# Autodesk Inventor assembly: shin_bracket_assem
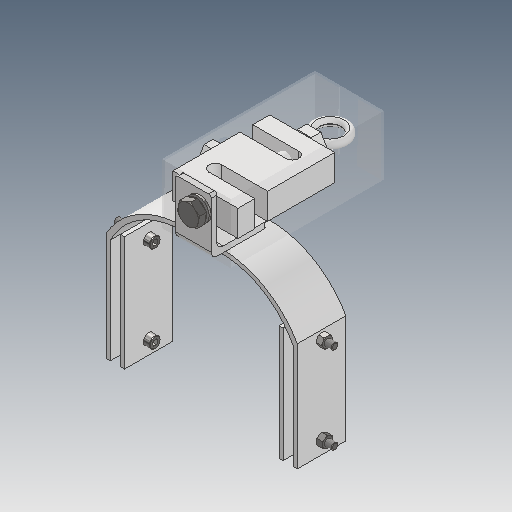
[picture p0: Inventor's stored thumbnail of the model, 512x512]
Saved by Autodesk Inventor 2025.2 (Build 292293000, 293)
## iProperties
Created: 2025-02-16
Part Number: shin_bracket_assem
Document SubType Name: Assembly
Designer: email
Author: email
## Documents named in this file (12)
- C:\Users\email\Desktop\Projects\Capstone\4TB6\CAD_Model\thigh_mount_2\shin_bracket_assem.iam
- C:\Users\email\Desktop\Projects\Capstone\4TB6\CAD_Model\thigh_mount_2\shin_bracket.ipt
- C:\Users\email\Desktop\Projects\Capstone\4TB6\CAD_Model\thigh_mount_2\shin_tab.ipt
- C:\Users\email\Documents\Inventor\Content Center Files\R2025\en-US\CSN 02 1143  A\CSN 02 1143 - M5 x 0.8 x 25(1).ipt
- C:\Users\email\Documents\Inventor\Content Center Files\R2025\en-US\AS 1112 (2)\AS 1112 - M5  Type 5.ipt
- C:\Users\email\Desktop\Projects\Capstone\4TB6\CAD_Model\thigh_mount_2\shin_L_bracket.ipt
- C:\Users\email\Documents\Inventor\Content Center Files\R2025\en-US\AS 1237 (2.1)\AS 1237 - 10.ipt
- C:\Users\email\Documents\Inventor\Content Center Files\R2025\en-US\AS 1110\AS 1110 - M10 x 16.ipt
- C:\Users\email\Documents\Inventor\Content Center Files\R2025\en-US\AS 1112 (2)\AS 1112 - M10  Type 5.ipt
- C:\Users\email\Desktop\Projects\Capstone\4TB6\CAD_Model\thigh_mount_2\tension_sensor_bolty.ipt
- C:\Users\email\Desktop\Projects\Capstone\4TB6\CAD_Model\thigh_mount_2\tension_sensor.ipt
- C:\Users\email\Desktop\Projects\Capstone\4TB6\CAD_Model\thigh_mount_2\tension_sensor_cover.ipt
## Components (21 placed, 11 different names)
1. shin_bracket:1 — Mate:2, Mate:3, Mate:11, Mate:12, Mate:13, Mate:14, Mate:19, Mate:20, Mate:21, Mate:22, Mate:23, Mate:24, Mate:26, Mate:28, Angle:1
2. shin_tab:1 — Mate:1, Mate:4, Mate:5, Mate:6, Mate:14
3. shin_tab:2 — Mate:7, Mate:8, Mate:9, Mate:10, Mate:13
4. CSN 02 1143 A M5 x 25:1 — Mate:1, Mate:2, Mate:5, Mate:17
5. CSN 02 1143 A M5 x 25:2 — Mate:3, Mate:4, Mate:6, Mate:18
6. CSN 02 1143 A M5 x 25:3 — Mate:7, Mate:9, Mate:11, Mate:15
7. CSN 02 1143 A M5 x 25:4 — Mate:8, Mate:10, Mate:12, Mate:16
8. AS 1112 (2) - Metric M5  Type 5:1 — Mate:16, Mate:20
9. AS 1112 (2) - Metric M5  Type 5:2 — Mate:15, Mate:19
10. AS 1112 (2) - Metric M5  Type 5:3 — Mate:17, Mate:21
11. AS 1112 (2) - Metric M5  Type 5:4 — Mate:18, Mate:22
12. shin_L_bracket:1 — Mate:23, Mate:24, Mate:30, Mate:31, Mate:32, Mate:33, Mate:36, Angle:1, Angle:2
13. AS 1237 (2.1) 10:1 — Mate:25, Mate:27, Mate:28
14. AS 1110 - Metric M10 x 16:1 — Mate:25, Mate:26, Mate:27, Mate:29
15. AS 1112 (2) - Metric M10  Type 5:1 — Mate:29, Mate:30
16. tension_sensor_bolty:1 — Mate:37, Mate:38, Mate:39
17. tension_sensor:1 — Mate:31, Mate:32, Mate:37, Mate:40, Angle:2
18. AS 1110 - Metric M10 x 16:2 — Mate:33, Mate:35, Mate:41, Mate:42
19. AS 1237 (2.1) 10:2 — Mate:35, Mate:36, Mate:43
20. AS 1237 (2.1) 10:3 — Mate:38, Mate:39, Mate:40
21. tension_sensor_cover:1 — Mate:41, Mate:42, Mate:43
## Relationships (44: Mate 42, Angle 2)
- Mate:1: shin_tab:1 ↔ CSN 02 1143 A M5 x 25:1
- Mate:2: shin_bracket:1 ↔ CSN 02 1143 A M5 x 25:1
- Mate:3: shin_bracket:1 ↔ CSN 02 1143 A M5 x 25:2
- Mate:4: shin_tab:1 ↔ CSN 02 1143 A M5 x 25:2
- Mate:5: shin_tab:1 ↔ CSN 02 1143 A M5 x 25:1
- Mate:6: shin_tab:1 ↔ CSN 02 1143 A M5 x 25:2
- Mate:7: shin_tab:2 ↔ CSN 02 1143 A M5 x 25:3
- Mate:8: shin_tab:2 ↔ CSN 02 1143 A M5 x 25:4
- Mate:9: shin_tab:2 ↔ CSN 02 1143 A M5 x 25:3
- Mate:10: shin_tab:2 ↔ CSN 02 1143 A M5 x 25:4
- Mate:11: shin_bracket:1 ↔ CSN 02 1143 A M5 x 25:3
- Mate:12: shin_bracket:1 ↔ CSN 02 1143 A M5 x 25:4
- Mate:13 (8 mm): shin_bracket:1 ↔ shin_tab:2
- Mate:14 (8 mm): shin_bracket:1 ↔ shin_tab:1
- Mate:15: CSN 02 1143 A M5 x 25:3 ↔ AS 1112 (2) - Metric M5  Type 5:2
- Mate:16: CSN 02 1143 A M5 x 25:4 ↔ AS 1112 (2) - Metric M5  Type 5:1
- Mate:17: CSN 02 1143 A M5 x 25:1 ↔ AS 1112 (2) - Metric M5  Type 5:3
- Mate:18: CSN 02 1143 A M5 x 25:2 ↔ AS 1112 (2) - Metric M5  Type 5:4
- Mate:19: shin_bracket:1 ↔ AS 1112 (2) - Metric M5  Type 5:2
- Mate:20: shin_bracket:1 ↔ AS 1112 (2) - Metric M5  Type 5:1
- Mate:21: shin_bracket:1 ↔ AS 1112 (2) - Metric M5  Type 5:3
- Mate:22: shin_bracket:1 ↔ AS 1112 (2) - Metric M5  Type 5:4
- Mate:23: shin_bracket:1 ↔ shin_L_bracket:1
- Mate:24: shin_bracket:1 ↔ shin_L_bracket:1
- Mate:25: AS 1237 (2.1) 10:1 ↔ AS 1110 - Metric M10 x 16:1
- Mate:26: shin_bracket:1 ↔ AS 1110 - Metric M10 x 16:1
- Mate:27: AS 1237 (2.1) 10:1 ↔ AS 1110 - Metric M10 x 16:1
- Mate:28: shin_bracket:1 ↔ AS 1237 (2.1) 10:1
- Mate:29: AS 1110 - Metric M10 x 16:1 ↔ AS 1112 (2) - Metric M10  Type 5:1
- Mate:30: shin_L_bracket:1 ↔ AS 1112 (2) - Metric M10  Type 5:1
- Mate:31: shin_L_bracket:1 ↔ tension_sensor:1
- Mate:32: shin_L_bracket:1 ↔ tension_sensor:1
- Mate:33: shin_L_bracket:1 ↔ AS 1110 - Metric M10 x 16:2
- Mate:35: AS 1110 - Metric M10 x 16:2 ↔ AS 1237 (2.1) 10:2
- Mate:36: shin_L_bracket:1 ↔ AS 1237 (2.1) 10:2
- Mate:37: tension_sensor_bolty:1 ↔ tension_sensor:1
- Mate:38: tension_sensor_bolty:1 ↔ AS 1237 (2.1) 10:3
- Mate:39: tension_sensor_bolty:1 ↔ AS 1237 (2.1) 10:3
- Mate:40: tension_sensor:1 ↔ AS 1237 (2.1) 10:3
- Angle:1 (0 deg): shin_bracket:1 ↔ shin_L_bracket:1
- Angle:2 (0 deg): shin_L_bracket:1 ↔ tension_sensor:1
- Mate:41: AS 1110 - Metric M10 x 16:2 ↔ tension_sensor_cover:1
- Mate:42: AS 1110 - Metric M10 x 16:2 ↔ tension_sensor_cover:1
- Mate:43: AS 1237 (2.1) 10:2 ↔ tension_sensor_cover:1
